# Autodesk Inventor assembly: Assembly1
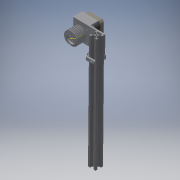
[picture p0: Inventor's stored thumbnail of the model, 180x180]
Saved by Autodesk Inventor 2019.4 (Build 234330000, 330)
## iProperties
Created: 2020-12-22
Part Number: Assembly1
Document SubType Name: Assembly
Designer: Jorian Brusind
Author: Jorian Brusind
## Documents named in this file (7)
- C:\Users\Jorian Brusind\Documents\GitHub\PersonalProjects\SpyderRobot\Inventor Files\Assembly1.iam
- C:\Users\Jorian Brusind\Documents\GitHub\PersonalProjects\SpyderRobot\Inventor Files\20 X 20 mm Extrusion 300mm.ipt
- C:\Users\Jorian Brusind\Documents\GitHub\PersonalProjects\SpyderRobot\Inventor Files\StepperMount.ipt
- C:\Users\Jorian Brusind\Documents\GitHub\PersonalProjects\SpyderRobot\Inventor Files\NEMA17 Motor Model\Nema 17  Stepper Motor length 34mm.ipt
- C:\Users\Jorian Brusind\Documents\GitHub\PersonalProjects\SpyderRobot\Inventor Files\Stepper_Coupler.ipt
- C:\Users\Jorian Brusind\Documents\GitHub\PersonalProjects\SpyderRobot\Inventor Files\Line_Spiral.ipt
- C:\Users\Jorian Brusind\Documents\GitHub\PersonalProjects\SpyderRobot\Inventor Files\Line_Guide.ipt
## Components (6 placed, 6 different names)
1. 20 X 20 mm Extrusion 300mm:1 — Mate:1, Flush:1, Mate:12, Mate:13, Mate:14
2. StepperMount:1 — Mate:1, Flush:1, Mate:3, Mate:4, Mate:6, Mate:12, Mate:15, Mate:16
3. Nema 17  Stepper Motor length 34mm:1 — Mate:3, Mate:4, Mate:5, Mate:16
4. Stepper_Coupler:1 — Mate:5, Mate:6, Mate:7, Mate:8, Mate:9
5. Line_Spiral:1 — Mate:7, Mate:8, Mate:9
6. Line_Guide:1 — Mate:13, Mate:14, Mate:15
## Relationships (14: Mate 13, Flush 1)
- Mate:1: 20 X 20 mm Extrusion 300mm:1 ↔ StepperMount:1
- Flush:1: 20 X 20 mm Extrusion 300mm:1 ↔ StepperMount:1
- Mate:3: StepperMount:1 ↔ Nema 17  Stepper Motor length 34mm:1
- Mate:4: StepperMount:1 ↔ Nema 17  Stepper Motor length 34mm:1
- Mate:5: Nema 17  Stepper Motor length 34mm:1 ↔ Stepper_Coupler:1
- Mate:6: StepperMount:1 ↔ Stepper_Coupler:1
- Mate:7: Stepper_Coupler:1 ↔ Line_Spiral:1
- Mate:8: Stepper_Coupler:1 ↔ Line_Spiral:1
- Mate:9: Stepper_Coupler:1 ↔ Line_Spiral:1
- Mate:12 (20 mm): 20 X 20 mm Extrusion 300mm:1 ↔ StepperMount:1
- Mate:13 (1 mm): 20 X 20 mm Extrusion 300mm:1 ↔ Line_Guide:1
- Mate:14: 20 X 20 mm Extrusion 300mm:1 ↔ Line_Guide:1
- Mate:15: StepperMount:1 ↔ Line_Guide:1
- Mate:16: StepperMount:1 ↔ Nema 17  Stepper Motor length 34mm:1
